# Autodesk Inventor assembly: Leadscrew Constraint Rear for 4040 - Assembly
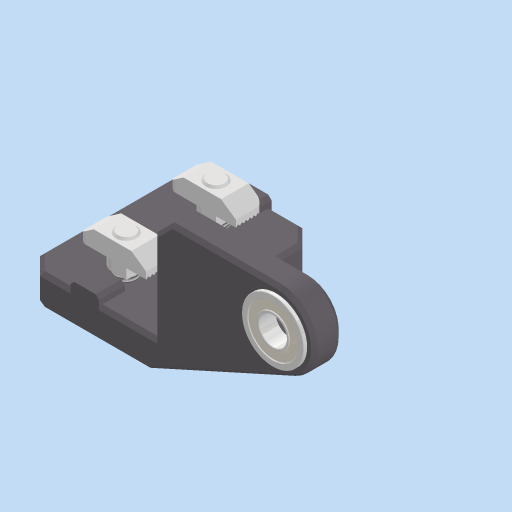
[picture p0: Inventor's stored thumbnail of the model, 512x512]
Saved by Autodesk Inventor 2023.2 (Build 272271000, 271)
## iProperties
Created: 2023-11-23
Part Number: Leadscrew Constraint Rear for 4040 - Assembly
Document SubType Name: Assembly
Designer: Nils Bade
Author: Nils Bade
## Documents named in this file (5)
- C:\Users\nilsb\Documents\Inventor\Projektarbeit-Bade\RatRig_modified\Leadscrew Constraint Rear for 4040 - Assembly.iam
- C:\Users\nilsb\Documents\Inventor\Projektarbeit-Bade\RatRig_modified\Leadscrew Constraint Rear for 4040.ipt
- C:\Users\nilsb\Documents\Inventor\Projektarbeit-Bade\RatRig_modified\T-NUT - DropIn 4040 SERIES - M6.ipt
- C:\Users\nilsb\Documents\Inventor\Projektarbeit-Bade\Schrauben\Cap Head Screw M6x16 - DIN912.ipt
- C:\Users\nilsb\Documents\Inventor\Projektarbeit-Bade\RatRig_Standards\Ball Bearing - F688ZZ v1.ipt
## Components (6 placed, 4 different names)
1. Leadscrew Constraint Rear 4040:1 — Passend:5, Passend:6, Passend:7, Passend:8, Passend:9, Passend:10, Winkel:1, Winkel:2, Passend:13, Passend:14
2. T-NUT - DROP IN TYPE FOR 40 SERIES - M6:1 — Passend:5, Passend:11, Winkel:1
3. T-NUT - DROP IN TYPE FOR 40 SERIES - M6:2 — Passend:6, Passend:12, Winkel:2
4. Cap Head Screw M6x16 - DIN912:1 — Passend:7, Passend:10, Passend:11
5. Cap Head Screw M6x16 - DIN912:2 — Passend:8, Passend:9, Passend:12
6. Ball Bearing - F688ZZ v1:1 — Passend:13, Passend:14
## Relationships (12: Mate 10, Angle 2)
- Passend:5 [Mate] (5.5 mm): Leadscrew Constraint Rear 4040:1 ↔ T-NUT - DROP IN TYPE FOR 40 SERIES - M6:1
- Passend:6 [Mate] (5.5 mm): Leadscrew Constraint Rear 4040:1 ↔ T-NUT - DROP IN TYPE FOR 40 SERIES - M6:2
- Passend:7 [Mate]: Leadscrew Constraint Rear 4040:1 ↔ Cap Head Screw M6x16 - DIN912:1
- Passend:8 [Mate]: Leadscrew Constraint Rear 4040:1 ↔ Cap Head Screw M6x16 - DIN912:2
- Passend:9 [Mate]: Leadscrew Constraint Rear 4040:1 ↔ Cap Head Screw M6x16 - DIN912:2
- Passend:10 [Mate]: Leadscrew Constraint Rear 4040:1 ↔ Cap Head Screw M6x16 - DIN912:1
- Passend:11 [Mate]: T-NUT - DROP IN TYPE FOR 40 SERIES - M6:1 ↔ Cap Head Screw M6x16 - DIN912:1
- Passend:12 [Mate]: T-NUT - DROP IN TYPE FOR 40 SERIES - M6:2 ↔ Cap Head Screw M6x16 - DIN912:2
- Winkel:1 [Angle] (0 deg): Leadscrew Constraint Rear 4040:1 ↔ T-NUT - DROP IN TYPE FOR 40 SERIES - M6:1
- Winkel:2 [Angle] (0 deg): Leadscrew Constraint Rear 4040:1 ↔ T-NUT - DROP IN TYPE FOR 40 SERIES - M6:2
- Passend:13 [Mate]: Leadscrew Constraint Rear 4040:1 ↔ Ball Bearing - F688ZZ v1:1
- Passend:14 [Mate]: Leadscrew Constraint Rear 4040:1 ↔ Ball Bearing - F688ZZ v1:1
